# Autodesk Inventor assembly: sprocket and bevel gear on shaft_MIR
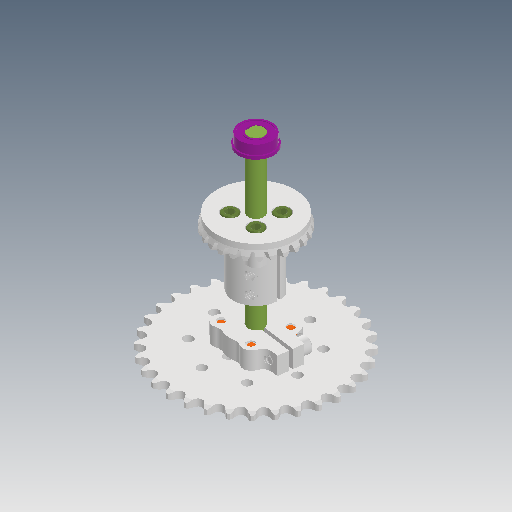
[picture p0: Inventor's stored thumbnail of the model, 512x512]
Saved by Autodesk Inventor 2020 (Build 240168000, 168)
## iProperties
Created: 2019-09-29
Part Number: sprocket and bevel gear on shaft_MIR
Document SubType Name: Assembly
Designer: ball
Author: ball
## Documents named in this file (6)
- C:\FTC\FTC8863CAD\2019 Robot\Mecanum Drive Train\sprocket and bevel gear on shaft_MIR.iam
- C:\FTC\FTC8863CAD\2019 Robot\Mecanum Drive Train\3_35 shaft_MIR.ipt
- C:\FTC\FTC8863CAD\2019 Robot\Mecanum Drive Train\bevel gear with clamping hub_MIR.iam
- C:\FTC\FTC8863CAD\2019 Robot\Mecanum Drive Train\32 spocket with hub_MIR.iam
- C:\FTC\FTC8863CAD\Actobotics\535 parts\535198_MIR.ipt
- C:\FTC\FTC8863CAD\Actobotics\633 parts\633104_MIR.ipt
## Components (8 placed, 5 different names)
1. 3_35 shaft_MIR:1 — Flush:3, Angle:1, Mate:7, Mate:6, Mate:4, Mate:1, Mate:16, Mate:12, Mate:14, Mate:15, Flush:4, Mate:17
2. bevel gear with clamping hub_MIR:1 [sub-assembly] — Flush:2, Mate:8, Mate:6, Mate:4
3. 32 spocket with hub_MIR:1 [sub-assembly] — Mate:8, Flush:3, Mate:1, Mate:13
4. 535198_MIR:1 — Mate:16, Mate:11
5. 633104_MIR:1 — Mate:13, Mate:12, Mate:9
6. 633104_MIR:2 — Mate:14, Mate:9, Mate:10
7. 633104_MIR:3 — Mate:15, Mate:11, Mate:10
8. 535198_MIR:2 — Flush:4, Mate:17
## Relationships (18: Mate 14, Flush 3, Angle 1)
- Flush:2: bevel gear with clamping hub_MIR:1
- Mate:8 (12.2174 mm): bevel gear with clamping hub_MIR:1 ↔ 32 spocket with hub_MIR:1
- Flush:3 (9.7028 mm): 3_35 shaft_MIR:1 ↔ 32 spocket with hub_MIR:1
- Angle:1 (90 deg): 3_35 shaft_MIR:1
- Mate:7: 3_35 shaft_MIR:1
- Mate:6: 3_35 shaft_MIR:1 ↔ bevel gear with clamping hub_MIR:1
- Mate:4: 3_35 shaft_MIR:1 ↔ bevel gear with clamping hub_MIR:1
- Mate:1: 3_35 shaft_MIR:1 ↔ 32 spocket with hub_MIR:1
- Mate:16: 3_35 shaft_MIR:1 ↔ 535198_MIR:1
- Mate:13: 32 spocket with hub_MIR:1 ↔ 633104_MIR:1
- Mate:12: 3_35 shaft_MIR:1 ↔ 633104_MIR:1
- Mate:14: 3_35 shaft_MIR:1 ↔ 633104_MIR:2
- Mate:9: 633104_MIR:1 ↔ 633104_MIR:2
- Mate:15: 3_35 shaft_MIR:1 ↔ 633104_MIR:3
- Mate:11: 535198_MIR:1 ↔ 633104_MIR:3
- Mate:10: 633104_MIR:2 ↔ 633104_MIR:3
- Flush:4: 3_35 shaft_MIR:1 ↔ 535198_MIR:2
- Mate:17: 3_35 shaft_MIR:1 ↔ 535198_MIR:2
